# Autodesk Inventor assembly: rocket_asm
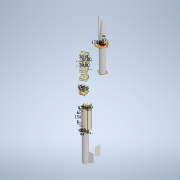
[picture p0: Inventor's stored thumbnail of the model, 180x180]
Saved by Autodesk Inventor 2020 (Build 240168000, 168)
## iProperties
Created: 2022-01-25
Part Number: rocket_asm
Document SubType Name: Assembly
Designer: sp
Author: sp
## Documents named in this file (13)
- C:\Users\sp\Documents\Rocket\rocket\CAD\rocket_asm.iam
- C:\Users\sp\Documents\Rocket\rocket\CAD\Segment_Engine.ipt
- C:\Users\sp\Documents\Rocket\rocket\CAD\Segment_mitte.ipt
- C:\Users\sp\Documents\Rocket\rocket\CAD\Segment_spitze.ipt
- C:\Users\sp\Documents\Rocket\rocket\CAD\Spitze.ipt
- C:\Users\sp\Documents\Rocket\rocket\CAD\Engine.ipt
- C:\Users\sp\Documents\Rocket\rocket\CAD\Leitwerk.ipt
- C:\Users\sp\Documents\Rocket\rocket\CAD\Back_holder.ipt
- C:\Users\sp\Documents\Rocket\rocket\CAD\Servo_Ku_asm.iam
- C:\Users\sp\Documents\Rocket\rocket\CAD\Elektro_asm.iam
- C:\Users\sp\Documents\Rocket\rocket\CAD\Ronde_Engine.ipt
- C:\Users\sp\Documents\Rocket\rocket\CAD\recovery_structure_asm.iam
- C:\Users\sp\Documents\Rocket\rocket\CAD\Cam_konstruction.ipt
## Components (14 placed, 12 different names)
1. Segment_Engine:1 — Einfügen:8
2. Segment_mitte:1 — Einfügen:6
3. Segment_spitze:1 — Passend:6, Einfügen:5
4. Spitze:1 — Einfügen:7
5. Engine:1 — Passend:6, Passend:8, Fluchtend:1, Passend:9, Passend:10, Passend:11, Fluchtend:2, Passend:12, Passend:13, Fluchtend:3, Passend:15, Passend:16, Passend:18, Einfügen:4
6. Leitwerk:1 — Passend:8, Fluchtend:1, Passend:9
7. Leitwerk:2 — Passend:10, Passend:11, Fluchtend:2
8. Leitwerk:3 — Passend:12, Passend:13, Fluchtend:3
9. Back_holder:1 — Passend:15, Passend:16
10. Servo_Ku_asm:1 [sub-assembly] — Einfügen:6
11. Elektro_asm:1 [sub-assembly]
12. Ronde_Engine:1 — Passend:18, Einfügen:4
13. recovery_structure_asm:1 [sub-assembly] — Einfügen:5
14. Cam_konstruction:1 — Einfügen:7, Einfügen:8
## Relationships (18: Mate 10, Insert 5, Flush 3)
- Passend:6 [Mate]: Segment_spitze:1 ↔ Engine:1
- Passend:8 [Mate]: Engine:1 ↔ Leitwerk:1
- Fluchtend:1 [Flush]: Engine:1 ↔ Leitwerk:1
- Passend:9 [Mate] (10.5 mm): Engine:1 ↔ Leitwerk:1
- Passend:10 [Mate]: Engine:1 ↔ Leitwerk:2
- Passend:11 [Mate]: Engine:1 ↔ Leitwerk:2
- Fluchtend:2 [Flush]: Engine:1 ↔ Leitwerk:2
- Passend:12 [Mate]: Engine:1 ↔ Leitwerk:3
- Passend:13 [Mate]: Engine:1 ↔ Leitwerk:3
- Fluchtend:3 [Flush]: Engine:1 ↔ Leitwerk:3
- Passend:15 [Mate]: Engine:1 ↔ Back_holder:1
- Passend:16 [Mate]: Engine:1 ↔ Back_holder:1
- Passend:18 [Mate]: Engine:1 ↔ Ronde_Engine:1
- Einfügen:4 [Insert]: Engine:1 ↔ Ronde_Engine:1
- Einfügen:5 [Insert]: Segment_spitze:1 ↔ recovery_structure_asm:1
- Einfügen:6 [Insert]: Segment_mitte:1 ↔ Servo_Ku_asm:1
- Einfügen:7 [Insert]: Spitze:1 ↔ Cam_konstruction:1
- Einfügen:8 [Insert]: Segment_Engine:1 ↔ Cam_konstruction:1
